# Autodesk Inventor assembly: 2.000 30A .500 With Adapters
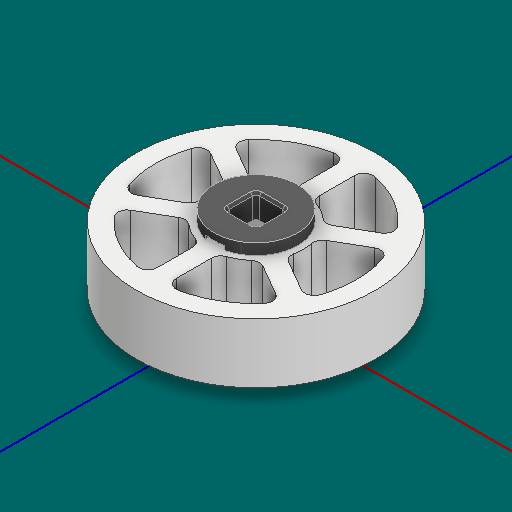
[picture p0: Inventor's stored thumbnail of the model, 512x512]
Saved by Autodesk Inventor 2025 (Build 290162000, 162)
## iProperties
Created: 2024-10-21
Part Number: 2.000 30A .500 With Adapters
Document SubType Name: Assembly
Designer: averey
Author: averey
## Documents named in this file (4)
- C:\Users\avere\VEX\High Stakes\CAD\ROBOPROS-CAD-Inventor\Quick Assemblies\2.000 30A .500 With Adapters.iam
- C:\Users\avere\VEX\High Stakes\CAD\ROBOPROS-CAD-Inventor\Motion\Wheels\Flex Wheels\2.000 Flex Wheel\2.000 30A .500.ipt
- C:\Users\avere\VEX\High Stakes\CAD\ROBOPROS-CAD-Inventor\Motion\Wheels\Flex Wheels\2.000 Flex Wheel.ipt
- C:\Users\avere\VEX\High Stakes\CAD\ROBOPROS-CAD-Inventor\Motion\Wheels\Flex Wheels\VersaHex Adapters .125.ipt
## Components (3 placed, 2 different names)
1. 2.000 30A .500:1 — Flush:1, Mate:1, Mate:2
2. VersaHex Adapters .125:1
3. VersaHex Adapters .125:2
## Relationships (5: Insert 2, Mate 2, Flush 1)
- [Insert]: 2.000 30A .500:1 ↔ VersaHex Adapters .125:1
- [Insert]: 2.000 30A .500:1 ↔ VersaHex Adapters .125:2
- Flush:1 (-6.35 mm): 2.000 30A .500:1
- Mate:1: 2.000 30A .500:1
- Mate:2: 2.000 30A .500:1
## Named parameters: d0_d1 = 0 mm
